# Autodesk Inventor assembly: linear_slider
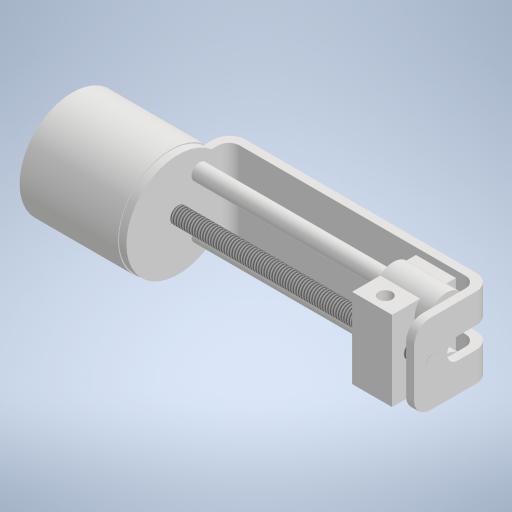
[picture p0: Inventor's stored thumbnail of the model, 512x512]
Saved by Autodesk Inventor 2024 (Build 280153000, 153)
## iProperties
Created: 2024-09-20
Part Number: linear_slider
Document SubType Name: Assembly
Designer: 1412z
Author: 1412z
## Documents named in this file (6)
- C:\Users\1412z\OneDrive\デスクトップ\研究室\農業ロボット\エンドエフェクタ\リニアガイドスライドテーブル\linear_slider.iam
- C:\Users\1412z\OneDrive\デスクトップ\研究室\農業ロボット\エンドエフェクタ\リニアガイドスライドテーブル\body.ipt
- C:\Users\1412z\OneDrive\デスクトップ\研究室\農業ロボット\エンドエフェクタ\リニアガイドスライドテーブル\stepping_motor.ipt
- C:\Users\1412z\OneDrive\デスクトップ\研究室\農業ロボット\エンドエフェクタ\リニアガイドスライドテーブル\shaft_screw.ipt
- C:\Users\1412z\OneDrive\デスクトップ\研究室\農業ロボット\エンドエフェクタ\リニアガイドスライドテーブル\shaft.ipt
- C:\Users\1412z\OneDrive\デスクトップ\研究室\農業ロボット\エンドエフェクタ\リニアガイドスライドテーブル\moving_part.ipt
## Components (6 placed, 5 different names)
1. body:1 — メイト:1, メイト:2, メイト:3, メイト:4, メイト:5, メイト:6, メイト:7, メイト:8
2. stepping_motor:1 — メイト:1, メイト:2, メイト:3, メイト:9
3. shaft_screw:1 — メイト:4, メイト:5
4. shaft:1 — メイト:8, メイト:9, 円柱状:1
5. shaft:2 — メイト:6, メイト:7, 円柱状:2
6. moving_part:1 — 円柱状:1, 円柱状:2
## Relationships (11: Mate 9, CylindricalJoint 2)
- メイト:1 [Mate]: body:1 ↔ stepping_motor:1
- メイト:2 [Mate]: body:1 ↔ stepping_motor:1
- メイト:3 [Mate]: body:1 ↔ stepping_motor:1
- メイト:4 [Mate]: body:1 ↔ shaft_screw:1
- メイト:5 [Mate]: body:1 ↔ shaft_screw:1
- メイト:6 [Mate]: body:1 ↔ shaft:2
- メイト:7 [Mate]: body:1 ↔ shaft:2
- メイト:8 [Mate]: body:1 ↔ shaft:1
- メイト:9 [Mate]: stepping_motor:1 ↔ shaft:1
- 円柱状:1 [CylindricalJoint]: shaft:1 ↔ moving_part:1
- 円柱状:2 [CylindricalJoint]: shaft:2 ↔ moving_part:1
